# Autodesk Inventor assembly: HB_armMountU03
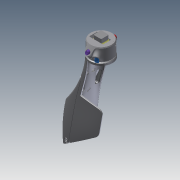
[picture p0: Inventor's stored thumbnail of the model, 180x180]
Saved by Autodesk Inventor 2015 SP1 (Build 190203100, 203)
## iProperties
Created: 2015-02-09
Part Number: HB_armMountU03
Document SubType Name: Assembly
Designer: Yamaura
Author: Yamaura
## Documents named in this file (17)
- C:\Users\Yamaura\Documents\GitHub\HACKberry\HACKberry-hardware\3D\Inventor\Parts\HB_armMountU03.iam
- C:\Users\Yamaura\Documents\GitHub\HACKberry\HACKberry-hardware\3D\Inventor\Parts\SBI-SUJ-1d4.ipt
- C:\Users\Yamaura\Documents\GitHub\HACKberry\HACKberry-hardware\3D\Inventor\Parts\CP 0.5-6-8.ipt
- C:\Users\Yamaura\Documents\GitHub\HACKberry\HACKberry-hardware\3D\Inventor\Parts\HBpronationLockPin02.ipt
- C:\Users\Yamaura\Documents\GitHub\HACKberry\HACKberry-hardware\3D\Inventor\Parts\HBlockPlateHolder02.ipt
- C:\Users\Yamaura\Documents\GitHub\HACKberry\HACKberry-hardware\3D\Inventor\Parts\HBwristMount01 v7.ipt
- C:\Users\Yamaura\Documents\GitHub\HACKberry\HACKberry-hardware\3D\Inventor\Parts\HBabductionLever02.ipt
- C:\Users\Yamaura\Documents\GitHub\HACKberry\HACKberry-hardware\3D\Inventor\Parts\HBejectorLever02.ipt
- C:\Users\Yamaura\Documents\GitHub\HACKberry\HACKberry-hardware\3D\Inventor\Parts\HBarmMount02.ipt
- C:\Users\Yamaura\Google ドライブ\exiii\3D\150405HackBerry\00_Latest\HbMainFrame03.ipt
- C:\Users\Yamaura\Documents\GitHub\HACKberry\HACKberry-hardware\3D\Inventor\Parts\150404Morikawa.ipt
- C:\Users\Yamaura\Documents\GitHub\HACKberry\HACKberry-hardware\3D\Inventor\Parts\ScrewM3L8Btite.ipt
- C:\Users\Yamaura\Documents\GitHub\HACKberry\HACKberry-hardware\3D\Inventor\Parts\HBarmMountBaseCover03.ipt
- C:\Users\Yamaura\Documents\GitHub\HACKberry\HACKberry-hardware\3D\Inventor\Parts\HBarmMountBase03.ipt
- C:\Users\Yamaura\Documents\GitHub\HACKberry\HACKberry-hardware\3D\Inventor\Parts\HbSocketU02.iam
- C:\Users\Yamaura\Documents\GitHub\HACKberry\HACKberry-hardware\3D\Inventor\Parts\HbSocketU03.iam
- C:\Users\Yamaura\Documents\GitHub\HACKberry\HACKberry-hardware\3D\Inventor\Parts\flatScrewM2L6PHI3.3T1.3.ipt
## Components (21 placed, 16 different names)
1. flatScrewM2L6PHI3.3T1.3:1
2. flatScrewM2L6PHI3.3T1.3:2
3. SBI-SUJ-1d4:1
4. CP 0.5-6-8:1 — メイト:56, メイト:57
5. CP 0.5-6-8:2
6. CP 0.5-6-8:3
7. CP 0.5-6-8:4
8. HBpronationLockPin02:1
9. HBlockPlateHolder02:1 — メイト:4, メイト:5, メイト:6, メイト:78, メイト:79
10. HBwristMount01 v7:1
11. HBarmMountBaseCover03:1 — メイト:74, メイト:75, 角度:4
12. HbMainFrame03:1 — メイト:3, メイト:4, メイト:5, メイト:6, 角度:1
13. HBabductionLever02:1 — メイト:41, 角度:2, メイト:56
14. HBejectorLever02:1 — メイト:57
15. HBarmMount02:1
16. 150404Morikawa:1
17. ScrewM3L8Btite:1
18. ScrewM3L8Btite:2
19. HBarmMountBase03:1 — メイト:76, フラッシュ:14, メイト:77
20. HbSocketU02:1 [sub-assembly] — フラッシュ:15, フラッシュ:16, フラッシュ:17
21. HbSocketU03:1 [sub-assembly] — メイト:77, メイト:78, メイト:79
## Relationships (20: Mate 13, Flush 4, Angle 3)
- メイト:3 [Mate]: HbMainFrame03:1
- メイト:4 [Mate]: HBlockPlateHolder02:1 ↔ HbMainFrame03:1
- メイト:5 [Mate]: HBlockPlateHolder02:1 ↔ HbMainFrame03:1
- メイト:6 [Mate]: HBlockPlateHolder02:1 ↔ HbMainFrame03:1
- 角度:1 [Angle] (90 deg): HbMainFrame03:1
- メイト:41 [Mate]: HBabductionLever02:1
- 角度:2 [Angle] (0 deg): HBabductionLever02:1
- メイト:56 [Mate]: CP 0.5-6-8:1 ↔ HBabductionLever02:1
- メイト:57 [Mate]: CP 0.5-6-8:1 ↔ HBejectorLever02:1
- メイト:74 [Mate]: HBarmMountBaseCover03:1
- メイト:75 [Mate] (9.2 mm): HBarmMountBaseCover03:1
- 角度:4 [Angle] (0 deg): HBarmMountBaseCover03:1
- メイト:76 [Mate]: HBarmMountBase03:1
- フラッシュ:14 [Flush] (-9.2 mm): HBarmMountBase03:1
- フラッシュ:15 [Flush]: HbSocketU02:1
- フラッシュ:16 [Flush]: HbSocketU02:1
- フラッシュ:17 [Flush]: HbSocketU02:1
- メイト:77 [Mate]: HBarmMountBase03:1 ↔ HbSocketU03:1
- メイト:78 [Mate]: HBlockPlateHolder02:1 ↔ HbSocketU03:1
- メイト:79 [Mate]: HBlockPlateHolder02:1 ↔ HbSocketU03:1
